# Autodesk Inventor assembly: 276-2016
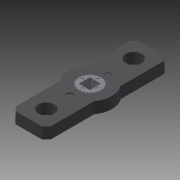
[picture p0: Inventor's stored thumbnail of the model, 180x180]
Saved by Autodesk Inventor 2016 SP2 (Build 200236200, 236)
## iProperties
Company: Autodesk Inc.
Category: Motion
Created: 2012-04-11
Part Number: 276-2016
Document SubType Name: Assembly
Designer: Autodesk Inc.
Catalog Web Link: http://www.vexrobotics.com/276-2016.html
Vendor: VEX
Author: Autodesk Inc.
## Documents named in this file (3)
- D:\Users\Owner\Desktop\Inventor Files\VEX Parts\Imperial\Motion\Lock Bar.iam
- D:\Users\Owner\Desktop\Inventor Files\VEX Parts\Imperial\Motion\Components\Shaft Lock Bar.ipt
- D:\Users\Owner\Desktop\Inventor Files\VEX Parts\Imperial\Motion\Components\Shaft Lock Bar Insert.ipt
## Components (2 placed, 2 different names)
1. Shaft Lock Bar:1 — Flush:1
2. Shaft Lock Bar Insert:1 — Flush:1
## Relationships (1: Flush 1)
- Flush:1: Shaft Lock Bar:1 ↔ Shaft Lock Bar Insert:1
